# Autodesk Inventor assembly: VatWithHolder
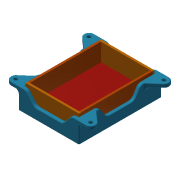
[picture p0: Inventor's stored thumbnail of the model, 180x180]
Saved by Autodesk Inventor 2014 (Build 180170000, 170)
## iProperties
Created: 2014-09-08
Part Number: VatWithHolder
Document SubType Name: Assembly
Designer: Peele
Author: Peele
## Documents named in this file (5)
- E:\Copy\DLP\PandaPrint\SubAssem\VatWithHolder.iam
- E:\Copy\DLP\PandaPrint\StockParts\BoroBottom.ipt
- E:\Copy\DLP\PandaPrint\StockParts\BoroSideLong.ipt
- E:\Copy\DLP\PandaPrint\StockParts\BoroSideShort.ipt
- E:\Copy\DLP\PandaPrint\CustomParts\VatHolder.ipt
## Components (6 placed, 4 different names)
1. BoroBottom:1 — Mate:1, Mate:2, Mate:3, Mate:4, Flush:1, Flush:2, Mate:5, Flush:3, Flush:4, Mate:8
2. BoroSideLong:1 — Mate:4, Flush:1, Flush:2
3. BoroSideLong:2 — Mate:5, Flush:3, Flush:4, Mate:6, Flush:5, Flush:6, Mate:7, Flush:7, Flush:8
4. BoroSideShort:1 — Mate:6, Flush:5, Flush:6
5. BoroSideShort:2 — Mate:7, Flush:7, Flush:8
6. VatHolder:1 — Mate:8, Mate:9, Mate:10
## Relationships (18: Mate 10, Flush 8)
- Mate:1: BoroBottom:1
- Mate:2: BoroBottom:1
- Mate:3: BoroBottom:1
- Mate:4: BoroBottom:1 ↔ BoroSideLong:1
- Flush:1: BoroBottom:1 ↔ BoroSideLong:1
- Flush:2: BoroBottom:1 ↔ BoroSideLong:1
- Mate:5: BoroBottom:1 ↔ BoroSideLong:2
- Flush:3: BoroBottom:1 ↔ BoroSideLong:2
- Flush:4: BoroBottom:1 ↔ BoroSideLong:2
- Mate:6: BoroSideLong:2 ↔ BoroSideShort:1
- Flush:5: BoroSideLong:2 ↔ BoroSideShort:1
- Flush:6: BoroSideLong:2 ↔ BoroSideShort:1
- Mate:7: BoroSideLong:2 ↔ BoroSideShort:2
- Flush:7: BoroSideLong:2 ↔ BoroSideShort:2
- Flush:8: BoroSideLong:2 ↔ BoroSideShort:2
- Mate:8: BoroBottom:1 ↔ VatHolder:1
- Mate:9: VatHolder:1
- Mate:10: VatHolder:1
